# Autodesk Inventor assembly: worm_gear
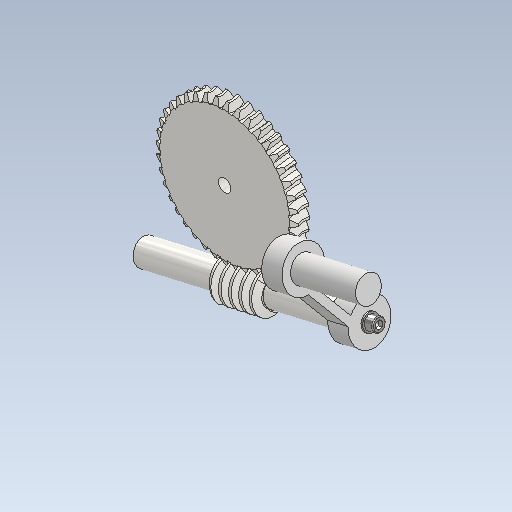
[picture p0: Inventor's stored thumbnail of the model, 512x512]
Saved by Autodesk Inventor 2020 (Build 240168000, 168)
## iProperties
Created: 2020-05-17
Part Number: worm_gear
Document SubType Name: Assembly
Designer: Hesekiel
Author: Hesekiel
## Documents named in this file (6)
- C:\Users\Hesekiel\Desktop\Equatorial-Mount-MUM\Mechanika\Mechanizm elewacji Filip\CAD\worm_gear.iam
- C:\Users\Hesekiel\Desktop\Equatorial-Mount-MUM\Mechanika\Mechanizm elewacji Filip\CAD\worm_gear\Design Accelerator\Worm Gears1.iam
- C:\Users\Hesekiel\Desktop\Equatorial-Mount-MUM\Mechanika\Mechanizm elewacji Filip\CAD\ramię_korby.ipt
- C:\Users\Hesekiel\Desktop\Equatorial-Mount-MUM\Mechanika\Mechanizm elewacji Filip\CAD\rączka_korby.ipt
- C:\Users\Hesekiel\Desktop\Equatorial-Mount-MUM\Mechanika\Mechanizm elewacji Filip\CAD\worm_gear\Design Accelerator\Bolted Connection1.iam
- C:\Users\Hesekiel\Desktop\Equatorial-Mount-MUM\Mechanika\Mechanizm elewacji Filip\CAD\worm_gear\Design Accelerator\Bolted Connection2.iam
## Components (5 placed, 4 different names)
1. Worm Gears:1 [sub-assembly] — Rigid:1
2. ramię_korby:1 — Rigid:1, Rigid:2, Mate:1, Mate:2, Mate:3, Mate:4
3. rączka_korby:1 — Rigid:2
4. Bolted Connection:1 [sub-assembly] — Mate:1, Mate:2
5. Bolted Connection:2 [sub-assembly] — Mate:3, Mate:4
## Relationships (6: Mate 4, WeldJoint 2)
- Rigid:1 [WeldJoint]: Worm Gears:1 ↔ ramię_korby:1
- Rigid:2 [WeldJoint]: ramię_korby:1 ↔ rączka_korby:1
- Mate:1: ramię_korby:1 ↔ Bolted Connection:1
- Mate:2: ramię_korby:1 ↔ Bolted Connection:1
- Mate:3: ramię_korby:1 ↔ Bolted Connection:2
- Mate:4: ramię_korby:1 ↔ Bolted Connection:2
